# Autodesk Inventor assembly: arm_assembly
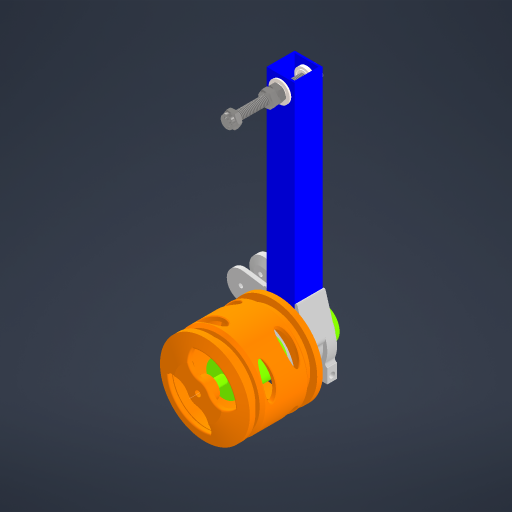
[picture p0: Inventor's stored thumbnail of the model, 512x512]
Saved by Autodesk Inventor 2024 (Build 280153000, 153)
## iProperties
Created: 2023-09-26
Part Number: arm_assembly
Document SubType Name: Assembly
Designer: user
Author: user
## Documents named in this file (9)
- D:\Docs\Robot\3d_v2\machine_body\arm_assembly_r.iam
- D:\Docs\Robot\3d_v2\base\arm.ipt
- D:\Docs\Robot\3d_v2\machine_body\arm_assembly\motor_holder.ipt
- D:\Docs\Robot\3d_v2\machine_body\arm_assembly\wheel.ipt
- D:\Docs\Robot\3d_v2\default_components\motor.ipt
- D:\Docs\Robot\3d_v2\default_components\F686zz.iam
- C:\Users\user\Documents\Inventor\Content Center Files\R2024\ru-RU\DIN 934\DIN 934 - M6 x 1.ipt
- C:\Users\user\Documents\Inventor\Content Center Files\R2024\ru-RU\DIN 933\DIN 933 - M6  x 60.ipt
- C:\Users\user\Documents\Inventor\Content Center Files\R2024\ru-RU\DIN 985\DIN 985 - M6.ipt
## Components (10 placed, 8 different names)
1. arm:1 — Совмещение:1, Совмещение:2, Совмещение:3, Совмещение:4, Совмещение:5, Совмещение:6, Совмещение:8, Вставка:2, Вставка:3
2. wheel:2 — Вставка:1, Совмещение:8
3. motor:1 — Совмещение:7, Вставка:1
4. motor_holder:1 — Совмещение:4, Совмещение:5, Совмещение:6, Совмещение:7
5. F686zz:1 [sub-assembly] — Вставка:3, Вставка:6
6. F686zz:2 [sub-assembly] — Вставка:2, Вставка:7
7. DIN 934 - заменено на DIN EN 24032/28673/28674 M6:1 — Вставка:5
8. DIN 934 - заменено на DIN EN 24032/28673/28674 M6:2 — Вставка:5, Вставка:7
9. DIN 933 - заменено на DIN EN 24017 M6  x 60:1 — Вставка:6, Вставка:8
10. DIN 985 - заменено на DIN EN ISO 10511 M6:1 — Вставка:8
## Relationships (15: Mate 8, Insert 7)
- Совмещение:1 [Mate]: arm:1
- Совмещение:2 [Mate]: arm:1
- Совмещение:3 [Mate]: arm:1
- Совмещение:4 [Mate]: arm:1 ↔ motor_holder:1
- Совмещение:5 [Mate]: arm:1 ↔ motor_holder:1
- Совмещение:6 [Mate]: arm:1 ↔ motor_holder:1
- Совмещение:7 [Mate]: motor:1 ↔ motor_holder:1
- Вставка:1 [Insert]: wheel:2 ↔ motor:1
- Совмещение:8 [Mate] (2 mm): arm:1 ↔ wheel:2
- Вставка:2 [Insert]: arm:1 ↔ F686zz:2
- Вставка:3 [Insert]: arm:1 ↔ F686zz:1
- Вставка:5 [Insert]: DIN 934 - заменено на DIN EN 24032/28673/28674 M6:1 ↔ DIN 934 - заменено на DIN EN 24032/28673/28674 M6:2
- Вставка:6 [Insert]: F686zz:1 ↔ DIN 933 - заменено на DIN EN 24017 M6  x 60:1
- Вставка:7 [Insert]: F686zz:2 ↔ DIN 934 - заменено на DIN EN 24032/28673/28674 M6:2
- Вставка:8 [Insert]: DIN 933 - заменено на DIN EN 24017 M6  x 60:1 ↔ DIN 985 - заменено на DIN EN ISO 10511 M6:1
